# Autodesk Inventor assembly: RightFootUnit
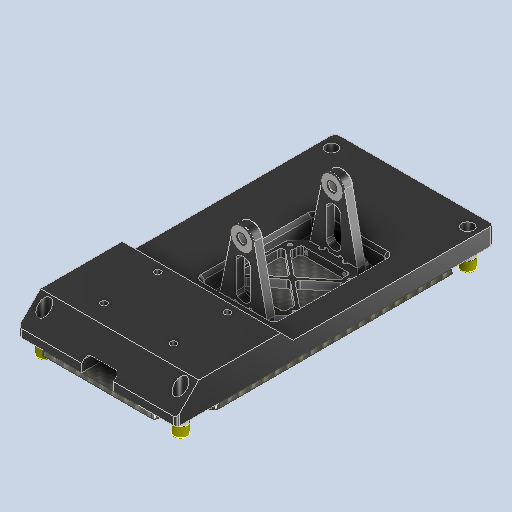
[picture p0: Inventor's stored thumbnail of the model, 512x512]
Saved by Autodesk Inventor 2024.2 (Build 282272000, 272)
## iProperties
Created: 2024-01-07
Part Number: RightFootUnit
Document SubType Name: Assembly
Designer: Masato Kubotera
Mass: 224.174 g
Surface Area: 1225.51 cm^2
Volume: 154.973 cm^3
Density: 1.44653 g/cm^3
Author: Masato Kubotera
## Documents named in this file (13)
- D:\OneDrive - Chiba Institute of Technology\CIT Brains\RoboCup2024\Mechanic\SUSTAINA-OP2\NativeFiles\Boby\LowerLimb\Feet\RightFootUnit.iam
- D:\OneDrive - Chiba Institute of Technology\CIT Brains\RoboCup2024\Mechanic\SUSTAINA-OP2\NativeFiles\Boby\LowerLimb\LegRollSliderFrame.ipt
- D:\OneDrive - Chiba Institute of Technology\CIT Brains\RoboCup2024\Mechanic\SUSTAINA-OP2\NativeFiles\Boby\COTS\Bushes\GFM-0608-06.ipt
- D:\OneDrive - Chiba Institute of Technology\CIT Brains\RoboCup2024\Mechanic\SUSTAINA-OP2\NativeFiles\Boby\COTS\Washers\Metal\UUW-0614-05H.ipt
- D:\OneDrive - Chiba Institute of Technology\CIT Brains\RoboCup2024\Mechanic\SUSTAINA-OP2\NativeFiles\Boby\COTS\Screws\CapScrew\UC-0310.ipt
- D:\OneDrive - Chiba Institute of Technology\CIT Brains\RoboCup2024\Mechanic\SUSTAINA-OP2\NativeFiles\Boby\LowerLimb\Feet\FootBraceFrame.ipt
- D:\OneDrive - Chiba Institute of Technology\CIT Brains\RoboCup2024\Mechanic\SUSTAINA-OP2\NativeFiles\Boby\LowerLimb\Feet\FootSoleFrame.ipt
- D:\OneDrive - Chiba Institute of Technology\CIT Brains\RoboCup2024\Mechanic\SUSTAINA-OP2\NativeFiles\Boby\COTS\Screws\CapScrew\UC-0308.ipt
- D:\OneDrive - Chiba Institute of Technology\CIT Brains\RoboCup2024\Mechanic\SUSTAINA-OP2\NativeFiles\Boby\COTS\MisumiComponents\URLM8.iam
- D:\OneDrive - Chiba Institute of Technology\CIT Brains\RoboCup2024\Mechanic\SUSTAINA-OP2\NativeFiles\Boby\COTS\ElectronicComponents\SC700-40kg.ipt
- D:\OneDrive - Chiba Institute of Technology\CIT Brains\RoboCup2024\Mechanic\SUSTAINA-OP2\NativeFiles\Boby\LowerLimb\Feet\RightFootCover.ipt
- D:\OneDrive - Chiba Institute of Technology\CIT Brains\RoboCup2024\Mechanic\SUSTAINA-OP2\NativeFiles\Boby\CustomElectronicComponents\Quad-Load-Cell-Amplifier-to-RS-485-Conv-Module.ipt
- D:\OneDrive - Chiba Institute of Technology\CIT Brains\RoboCup2024\Mechanic\SUSTAINA-OP2\NativeFiles\Boby\COTS\Washers\Resin\TT-0614-05.ipt
## Components (36 placed, 12 different names)
1. LegRollSliderFrame:1 — Mate:1, Angle:1, Flush:2, Flush:3, Insert:1, Insert:3, Insert:7, Insert:8, Insert:11, Insert:12, Mate:2
2. LegRollSliderFrame:2 — Flush:2, Flush:3, Insert:2, Insert:4, Insert:9, Insert:10, Insert:13, Insert:14
3. FootBraceFrame:1 — Insert:11, Insert:12, Insert:13, Insert:14, Insert:15, Insert:16, Insert:17, Insert:18
4. FootSoleFrame:1 — Insert:15, Insert:16, Insert:17, Insert:18, Insert:19, Insert:20, Insert:21, Insert:22, Insert:23, Insert:24, Insert:25, Insert:26, Insert:27, Insert:28, Insert:29, Insert:30, Insert:37, Insert:38, Insert:39, Insert:40, Insert:41, Insert:42, Insert:43, Insert:44, Flush:4, Mate:3, Mate:4
5. Quad-Load-Cell-Amplifier-to-RS-485-Conv-Module:1 — Insert:35, Insert:36
6. RightFootCover:1 — Insert:35, Insert:36, Flush:4, Mate:3, Mate:4
7. GFM-0608-06:1 — Insert:1
8. GFM-0608-06:2 — Insert:2
9. SC700-40kg:1 — Insert:23, Insert:24, Insert:31
10. SC700-40kg:2 — Insert:25, Insert:26, Insert:32
11. SC700-40kg:3 — Insert:27, Insert:28, Insert:33
12. SC700-40kg:4 — Insert:29, Insert:30, Insert:34
13. UC-0308:5 — Insert:41
14. UC-0310:5 — Insert:37
15. UC-0308:6 — Insert:42
16. UC-0310:6 — Insert:38
17. UC-0308:7 — Insert:43
18. UC-0310:7 — Insert:39
19. UC-0308:8 — Insert:44
20. UC-0310:8 — Insert:40
21. UC-0310:1 — Insert:7
22. UC-0310:2 — Insert:8
23. UC-0310:3 — Insert:9
24. UC-0310:4 — Insert:10
25. UC-0308:1 — Insert:19
26. UC-0308:2 — Insert:20
27. UC-0308:3 — Insert:21
28. UC-0308:4 — Insert:22
29. URLM8:1 [sub-assembly] — Insert:31
30. URLM8:2 [sub-assembly] — Insert:32
31. URLM8:3 [sub-assembly] — Insert:33
32. URLM8:4 [sub-assembly] — Insert:34
33. TT-0614-05:1 — Insert:3, Insert:5
34. TT-0614-05:2 — Insert:4, Insert:6
35. UUW-0614-05H:1 — Insert:5
36. UUW-0614-05H:2 — Insert:6
## Relationships (52: Insert 44, Mate 4, Flush 3, Angle 1)
- Mate:1: LegRollSliderFrame:1
- Angle:1 (180 deg): LegRollSliderFrame:1
- Flush:2: LegRollSliderFrame:1 ↔ LegRollSliderFrame:2
- Flush:3: LegRollSliderFrame:1 ↔ LegRollSliderFrame:2
- Insert:1: LegRollSliderFrame:1 ↔ GFM-0608-06:1
- Insert:2: LegRollSliderFrame:2 ↔ GFM-0608-06:2
- Insert:3: LegRollSliderFrame:1 ↔ TT-0614-05:1
- Insert:4: LegRollSliderFrame:2 ↔ TT-0614-05:2
- Insert:5: TT-0614-05:1 ↔ UUW-0614-05H:1
- Insert:6: TT-0614-05:2 ↔ UUW-0614-05H:2
- Insert:7: LegRollSliderFrame:1 ↔ UC-0310:1
- Insert:8: LegRollSliderFrame:1 ↔ UC-0310:2
- Insert:9: LegRollSliderFrame:2 ↔ UC-0310:3
- Insert:10: LegRollSliderFrame:2 ↔ UC-0310:4
- Insert:11: LegRollSliderFrame:1 ↔ FootBraceFrame:1
- Insert:12: LegRollSliderFrame:1 ↔ FootBraceFrame:1
- Insert:13: LegRollSliderFrame:2 ↔ FootBraceFrame:1
- Insert:14: LegRollSliderFrame:2 ↔ FootBraceFrame:1
- Mate:2 (16 mm): LegRollSliderFrame:1
- Insert:15: FootBraceFrame:1 ↔ FootSoleFrame:1
- Insert:16: FootBraceFrame:1 ↔ FootSoleFrame:1
- Insert:17: FootBraceFrame:1 ↔ FootSoleFrame:1
- Insert:18: FootBraceFrame:1 ↔ FootSoleFrame:1
- Insert:19: FootSoleFrame:1 ↔ UC-0308:1
- Insert:20: FootSoleFrame:1 ↔ UC-0308:2
- Insert:21: FootSoleFrame:1 ↔ UC-0308:3
- Insert:22: FootSoleFrame:1 ↔ UC-0308:4
- Insert:23: FootSoleFrame:1 ↔ SC700-40kg:1
- Insert:24: FootSoleFrame:1 ↔ SC700-40kg:1
- Insert:25: FootSoleFrame:1 ↔ SC700-40kg:2
- Insert:26: FootSoleFrame:1 ↔ SC700-40kg:2
- Insert:27: FootSoleFrame:1 ↔ SC700-40kg:3
- Insert:28: FootSoleFrame:1 ↔ SC700-40kg:3
- Insert:29: FootSoleFrame:1 ↔ SC700-40kg:4
- Insert:30: FootSoleFrame:1 ↔ SC700-40kg:4
- Insert:31: SC700-40kg:1 ↔ URLM8:1
- Insert:32: SC700-40kg:2 ↔ URLM8:2
- Insert:33: SC700-40kg:3 ↔ URLM8:3
- Insert:34: SC700-40kg:4 ↔ URLM8:4
- Insert:35: Quad-Load-Cell-Amplifier-to-RS-485-Conv-Module:1 ↔ RightFootCover:1
- Insert:36: Quad-Load-Cell-Amplifier-to-RS-485-Conv-Module:1 ↔ RightFootCover:1
- Insert:37: FootSoleFrame:1 ↔ UC-0310:5
- Insert:38: FootSoleFrame:1 ↔ UC-0310:6
- Insert:39: FootSoleFrame:1 ↔ UC-0310:7
- Insert:40: FootSoleFrame:1 ↔ UC-0310:8
- Insert:41: FootSoleFrame:1 ↔ UC-0308:5
- Insert:42: FootSoleFrame:1 ↔ UC-0308:6
- Insert:43: FootSoleFrame:1 ↔ UC-0308:7
- Insert:44: FootSoleFrame:1 ↔ UC-0308:8
- Flush:4: FootSoleFrame:1 ↔ RightFootCover:1
- Mate:3: FootSoleFrame:1 ↔ RightFootCover:1
- Mate:4 (-3 mm): FootSoleFrame:1 ↔ RightFootCover:1
